# Autodesk Inventor assembly: Arm 2.0 Assembly
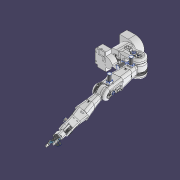
[picture p0: Inventor's stored thumbnail of the model, 180x180]
Saved by Autodesk Inventor 2017 SP1 (Build 210196100, 196)
## iProperties
Created: 2017-09-28
Part Number: Arm 2.0 Assembly
Document SubType Name: Assembly
Designer: Zach
Author: Zach
## Documents named in this file (62)
- C:\Users\Zach\Documents\GitHub\tr1\src\Body\Arm 2.0 Assembly\Arm 2.0 Assembly.iam
- C:\Users\Zach\Documents\GitHub\tr1\src\Body\Arm 2.0 Assembly\Steel Rod 8mm x 135mm.ipt
- C:\Users\Zach\Documents\GitHub\tr1\lib\22x8x8mm Bearing.ipt
- C:\Users\Zach\Documents\GitHub\tr1\src\Body\Arm 2.0 Assembly\AA004.ipt
- C:\Users\Zach\Documents\GitHub\tr1\lib\QS12MM250\QS12MM250.ipt
- C:\Users\Zach\Documents\GitHub\tr1\src\Body\Arm 2.0 Assembly\Steel Rod 8mm x 110mm.ipt
- C:\Users\Zach\Documents\GitHub\tr1\src\Body\Arm 2.0 Assembly\AA013.ipt
- C:\Users\Zach\Documents\GitHub\tr1\src\Body\Arm 2.0 Assembly\AA014.ipt
- C:\Users\Zach\Documents\GitHub\tr1\lib\12V DC Motor 378-1.ipt
- C:\Users\Zach\Documents\Inventor\Content Center Files\R2017\en-US\ISO 4017(1)\ISO 4017 - M5 x 20 - ISO.ipt
- C:\Users\Zach\Documents\GitHub\tr1\src\Body\Arm 2.0 Assembly\Steel Rod 8mm x 80mm.ipt
- C:\Users\Zach\Documents\GitHub\tr1\src\Body\Arm 2.0 Assembly\Gripper Assembly\Gripper B Assembly.iam
- C:\Users\Zach\Documents\GitHub\tr1\lib\8mm Hub.ipt
- C:\Users\Zach\Documents\GitHub\tr1\src\Body\Arm 2.0 Assembly\Arm 2.0 Assembly\Design Accelerator\Spur Gears5.iam
- C:\Users\Zach\Documents\GitHub\tr1\lib\4mm mounting hub.ipt
- C:\Users\Zach\Documents\GitHub\tr1\lib\6201RS\6201RS.ipt
- C:\Users\Zach\Documents\GitHub\tr1\lib\U51105\U51105.ipt
- C:\Users\Zach\Documents\GitHub\tr1\src\Body\Arm 2.0 Assembly\AA034.ipt
- C:\Users\Zach\Documents\GitHub\tr1\src\Body\Arm 2.0 Assembly\Arm 2.0 Assembly\Design Accelerator\Spur Gears6.iam
- C:\Users\Zach\Documents\GitHub\tr1\src\Body\Arm 2.0 Assembly\AA008c.ipt
- C:\Users\Zach\Documents\GitHub\tr1\src\Body\Arm 2.0 Assembly\Arm 2.0 Assembly\Design Accelerator\Spur Gears7.iam
- C:\Users\Zach\Documents\GitHub\tr1\src\Body\Arm 2.0 Assembly\AA036.ipt
- C:\Users\Zach\Documents\GitHub\tr1\src\Body\Arm 2.0 Assembly\AA037.ipt
- C:\Users\Zach\Documents\GitHub\tr1\src\Body\Arm 2.0 Assembly\AA016b.ipt
- C:\Users\Zach\Documents\GitHub\tr1\src\Body\Arm 2.0 Assembly\AA005b.ipt
- C:\Users\Zach\Documents\GitHub\tr1\src\Body\Arm 2.0 Assembly\AA006b.ipt
- C:\Users\Zach\Documents\GitHub\tr1\src\Body\Arm 2.0 Assembly\AA001c.ipt
- C:\Users\Zach\Documents\GitHub\tr1\src\Body\Arm 2.0 Assembly\Arm 2.0 Assembly\Design Accelerator\Spur Gears8.iam
- C:\Users\Zach\Documents\GitHub\tr1\src\Body\Arm 2.0 Assembly\Arm 2.0 Assembly\Design Accelerator\Spur Gears11.iam
- C:\Users\Zach\Documents\GitHub\tr1\src\Body\Arm 2.0 Assembly\Arm 2.0 Assembly\Design Accelerator\Spur Gears9.iam
- C:\Users\Zach\Documents\GitHub\tr1\src\Body\Arm 2.0 Assembly\AA010b.ipt
- C:\Users\Zach\Documents\GitHub\tr1\src\Body\Arm 2.0 Assembly\Arm 2.0 Assembly\Design Accelerator\Spur Gears10.iam
- C:\Users\Zach\Documents\GitHub\tr1\src\Body\Arm 2.0 Assembly\Arm 2.0 Assembly\Design Accelerator\Spur Gears12.iam
- C:\Users\Zach\Documents\GitHub\tr1\src\Body\Arm 2.0 Assembly\AA041.ipt
- C:\Users\Zach\Documents\Inventor\Content Center Files\R2017\en-US\ISO 7045  H\ISO 7045 - M3 x 8 - 4.8 - H - ISO.ipt
- C:\Users\Zach\Documents\GitHub\tr1\src\Body\Arm 2.0 Assembly\Arm 2.0 Assembly\Design Accelerator\Spur Gears13.iam
- C:\Users\Zach\Documents\GitHub\tr1\src\Body\Arm 2.0 Assembly\Arm 2.0 Assembly\Design Accelerator\Spur Gears16.iam
- C:\Users\Zach\Documents\GitHub\tr1\src\Body\Arm 2.0 Assembly\AA046.ipt
- C:\Users\Zach\Documents\GitHub\tr1\lib\MG995.ipt
- C:\Users\Zach\Documents\GitHub\tr1\lib\Servo Mounting Hub.ipt
- C:\Users\Zach\Documents\GitHub\tr1\src\Body\Arm 2.0 Assembly\AA047.ipt
- C:\Users\Zach\Documents\GitHub\tr1\src\Body\Arm 2.0 Assembly\AA048.ipt
- C:\Users\Zach\Documents\Inventor\Content Center Files\R2017\en-US\ISO 4018\ISO 4018 - M5 x 10.ipt
- C:\Users\Zach\Documents\Inventor\Content Center Files\R2017\en-US\ISO 4018\ISO 4018 - M5 x 25.ipt
- C:\Users\Zach\Documents\Inventor\Content Center Files\R2017\en-US\ISO 7045  H\ISO 7045 - M3 x 12 - 4.8 - H - ISO.ipt
- C:\Users\Zach\Documents\GitHub\tr1\src\Body\Arm 2.0 Assembly\AA049.ipt
- C:\Users\Zach\Documents\Inventor\Content Center Files\R2017\en-US\ISO 4018\ISO 4018 - M5 x 40.ipt
- C:\Users\Zach\Documents\Inventor\Content Center Files\R2017\en-US\ISO 4035(2)\ISO 4035 - M5 - ISO.ipt
- C:\Users\Zach\Documents\Inventor\Content Center Files\R2017\en-US\ISO 4018\ISO 4018 - M5 x 35.ipt
- C:\Users\Zach\Documents\Inventor\Content Center Files\R2017\en-US\ISO 4762(2)\ISO 4762 - M4 x 10ISO.ipt
- C:\Users\Zach\Documents\GitHub\tr1\src\Body\Arm 2.0 Assembly\AA050.ipt
- C:\Users\Zach\Documents\GitHub\tr1\lib\6mm Mounting Hub.ipt
- C:\Users\Zach\Documents\GitHub\tr1\src\Body\Arm 2.0 Assembly\AA035c.ipt
- C:\Users\Zach\Documents\GitHub\tr1\src\Body\Arm 2.0 Assembly\AA008d2.ipt
- C:\Users\Zach\Documents\GitHub\tr1\lib\TSINY TS-42GZ495.ipt
- C:\Users\Zach\Documents\GitHub\tr1\lib\EMS22XXX-D28-LSX.ipt
- C:\Users\Zach\Documents\GitHub\tr1\lib\6mm x 160mm D Shaft.ipt
- C:\Users\Zach\Documents\GitHub\tr1\src\Body\Arm 2.0 Assembly\AA051.ipt
- C:\Users\Zach\Documents\GitHub\tr1\src\Body\Arm 2.0 Assembly\AA052.ipt
- C:\Users\Zach\Documents\GitHub\tr1\src\Body\Arm 2.0 Assembly\AA045b.ipt
- C:\Users\Zach\Documents\GitHub\tr1\lib\6mm x 120mm D Shaft.ipt
- C:\Users\Zach\Documents\GitHub\tr1\src\Body\Arm 2.0 Assembly\AA053.ipt
## Components (215 placed, 61 different names)
1. AA001c:1 — Mate:554, Mate:555, Mate:556, Mate:560, Mate:562, Mate:563, Mate:564, Mate:565, Mate:566, Mate:567, Mate:576, Mate:578, Mate:581, Mate:592, Mate:602, Mate:895, Mate:905, Mate:906, Mate:1083, Mate:1084, Mate:1085, Mate:1086, Mate:1093, Angle:18, Mate:1095, Mate:1122, Mate:1261, Mate:1262, Mate:1263
2. AA004:1 — Mate:23, Mate:345, Mate:347, Mate:350, Mate:357, Mate:554, Mate:555, Mate:556, Mate:590, Mate:591, Mate:826
3. AA005b:1 — Mate:537, Mate:538, Mate:539, Mate:541, Mate:542, Mate:543, Mate:806, Mate:807, Mate:808, Mate:809, Mate:838, Mate:909, Mate:910
4. AA006b:1 — Mate:544, Mate:593, Mate:594, Mate:598, Mate:599, Mate:609, Mate:802, Mate:803, Mate:804, Mate:805, Mate:838, Mate:1088, Mate:1089, Angle:17, Mate:1233
5. AA008c:1 — Mate:451, Mate:616, Mate:1113, Mate:1114, Mate:1115, Mate:1125
6. AA008d2:1 — Mate:1104, Mate:1106, Mate:1107, Angle:22, Mate:1113, Mate:1114, Mate:1115, Mate:1124, Mate:1125, Mate:1157, Mate:1158, Mate:1159, Mate:1160, Mate:1161, Mate:1162, Mate:1163, Mate:1164, Mate:1165, Mate:1166, Mate:1170, Mate:1192, Mate:1193, Mate:1194, Mate:1195
7. AA010b:1 — Mate:616, Mate:620, Mate:621, Mate:624, Mate:625, Mate:626, Mate:628, Mate:630, Mate:642, Flush:20, Mate:648, Mate:650, Mate:948, Mate:1097, Mate:1098, Angle:21, Mate:1100, Mate:1101, Mate:1102, Mate:1126, Mate:1130, Mate:1152, Mate:1204, Mate:1237, Mate:1258, Mate:1259, Mate:1260
8. AA013:2 — Mate:142, Mate:143, Mate:144, Mate:145, Mate:146, Mate:147, Mate:563, Mate:564, Mate:565
9. AA014:2 — Mate:628, Mate:629, Mate:630, Mate:976, Mate:977, Mate:978, Mate:979, Mate:980, Mate:981
10. AA016b:1 — Mate:518, Mate:519, Mate:520, Mate:529, Mate:530, Mate:664, Mate:665, Mate:667, Mate:671, Mate:673, Mate:675, Mate:676, Mate:677, Mate:877, Mate:878, Mate:1206, Mate:1207, Angle:26
11. AA034:1 — Mate:529, Mate:534, Mate:535, Mate:879, Mate:880, Mate:881, Mate:882, Mate:883, Mate:884, Mate:885, Mate:886, Mate:964, Mate:965, Mate:966, Mate:967, Mate:968, Mate:969, Mate:970, Mate:971, Mate:972, Mate:973, Mate:974, Mate:975, Mate:1213, Mate:1256, Mate:1257
12. AA035c:1 — Mate:1076, Mate:1077, Mate:1167, Mate:1168, Mate:1169, Mate:1170, Mate:1171, Mate:1172, Mate:1173, Mate:1175, Angle:24, Angle:25, Mate:1176, Mate:1202, Mate:1203
13. AA036:1 — Mate:498, Mate:501, Mate:502, Mate:511, Mate:698, Mate:868, Mate:871, Mate:872, Mate:939, Mate:1197, Mate:1198, Mate:1199, Mate:1200
14. AA037:1 — Mate:501, Mate:502, Mate:514, Mate:515, Mate:516, Mate:518, Mate:519, Mate:520, Mate:530, Mate:664, Mate:665, Mate:698, Mate:866, Mate:867, Mate:873, Mate:874, Mate:875, Mate:876, Flush:25, Flush:26, Mate:950, Mate:951, Mate:952, Mate:953
15. AA041:1 — Mate:675, Mate:676, Mate:677, Mate:682, Mate:683, Mate:684, Mate:685, Mate:1250
16. AA045b:1 — Mate:1211, Mate:1212, Angle:27, Mate:1213, Mate:1214, Mate:1215, Mate:1216, Mate:1217, Mate:1218, Mate:1219, Flush:37, Mate:1221, Mate:1223, Mate:1224, Mate:1225, Mate:1227, Mate:1235, Mate:1264, Mate:1265
17. AA046:1 — Mate:727, Mate:728, Mate:731, Mate:735, Mate:736, Mate:737, Mate:752, Mate:756, Mate:757, Mate:758, Mate:759, Mate:760, Mate:761, Mate:762, Mate:763, Mate:1217
18. AA047:1 — Mate:735, Mate:736, Mate:737, Mate:738, Mate:739, Mate:740, Mate:753, Mate:754, Mate:755, Mate:800, Mate:801
19. AA048:1 — Mate:744, Mate:745, Mate:746, Mate:747, Mate:748, Mate:749
20. AA049:1 — Mate:783, Mate:786, Mate:787, Mate:788, Mate:789, Mate:790, Mate:791, Mate:1218
21. AA050:1 — Mate:994, Mate:995, Mate:999, Mate:1001, Mate:1002, Mate:1003, Mate:1004
22. AA051:1 — Mate:1196, Mate:1197
23. AA052:1 — Mate:1201, Mate:1202
24. AA053:1 — Mate:1258, Mate:1259, Mate:1260
25. AA053:3 — Mate:1261, Mate:1262, Mate:1263
26. Gripper B Assembly:1 [sub-assembly] — Mate:747, Mate:748, Mate:749
27. 22x8x8mm Bearing:1 — Mate:433, Mate:560
28. 22x8x8mm Bearing:2 — Mate:437, Mate:562
29. 22x8x8mm Bearing:3 — Mate:57, Mate:620, Mate:626
30. 22x8x8mm Bearing:4 — Mate:621, Mate:629, Mate:642
31. 22x8x8mm Bearing:5 — Mate:186, Mate:1265
32. 22x8x8mm Bearing:6 — Mate:187, Mate:1264
33. 22x8x8mm Bearing:7 — Mate:1247
34. 22x8x8mm Bearing:13 — Mate:451
35. QS12MM250:1 — Mate:23, Mate:344, Mate:346, Mate:348, Mate:354, Mate:537, Mate:544, Mate:593, Mate:594, Mate:597, Mate:1230
36. Steel Rod 8mm x 140mm:1 — Mate:433, Mate:437, Mate:476, Mate:575, Mate:651, Mate:1076, Mate:1122, Flush:35, Mate:1201
37. Steel Rod 8mm x 110mm:1 — Mate:57, Mate:491, Mate:498, Flush:20, Mate:649, Mate:1196, Mate:1204
38. Steel Rod 8mm x 80mm:1 — Mate:186, Mate:187, Mate:710, Mate:721, Mate:724, Mate:730, Mate:783, Mate:1216, Flush:37, Mate:1234
39. TSINY TS-42GZ495:3 — Mate:1104, Mate:1117, Mate:1135, Mate:1160, Mate:1161
40. TSINY TS-42GZ495:2 — Mate:1097, Mate:1098, Mate:1101, Mate:1102, Mate:1128, Mate:1129
41. TSINY TS-42GZ495:1 — Mate:1083, Mate:1084, Mate:1085, Mate:1086, Mate:1087
42. 12V DC Motor 378-1:3 — Mate:712, Mate:714, Mate:778, Mate:779, Mate:1224, Mate:1225
43. 12V DC Motor 378-1:4 — Mate:514, Mate:515, Mate:516, Mate:522
44. 12V DC Motor 378-1:6 — Mate:340, Mate:342, Mate:538, Mate:539, Mate:540, Mate:543, Mate:907, Mate:908
45. 6201RS:1 — Mate:346, Mate:347
46. 6201RS:2 — Mate:357, Mate:597
47. U51105:1 — Mate:348, Mate:349, Mate:542
48. U51105:2 — Mate:354, Mate:608, Mate:609, Mate:600
49. 6mm Mounting Hub:1 — Mate:1067, Mate:1069, Mate:1117, Mate:1136, Mate:1138, Mate:1139, Mate:1140, Flush:29, Mate:1243, Mate:1244
50. 6mm Mounting Hub:9 — Mate:1208, Flush:36, Mate:1209
51. 6mm Mounting Hub:7 — Mate:1185, Mate:1186, Mate:1188
52. 6mm Mounting Hub:8 — Mate:1189, Mate:1191
53. 6mm Mounting Hub:6 — Mate:1181, Mate:1183, Mate:1184
54. 6mm Mounting Hub:5 — Mate:1177, Mate:1178, Mate:1179
55. 6mm Mounting Hub:4 — Mate:1147, Mate:1148, Mate:1150, Mate:1152, Mate:1236, Mate:1238, Mate:1239, Mate:1240, Mate:1241, Mate:1242
56. 6mm Mounting Hub:2 — Mate:1090, Mate:1091
57. 8mm Hub:2 — Mate:534, Mate:535, Mate:1249, Mate:1254, Mate:1255
58. 8mm Hub:4 — Mate:580, Mate:581, Mate:582, Flush:35
59. 8mm Hub:6 — Mate:651, Mate:911, Mate:912, Mate:913, Mate:914, Mate:915, Mate:916, Mate:1203
60. 8mm Hub:7 — Mate:667, Mate:674, Flush:36, Mate:1248
61. 8mm Hub:8 — Mate:721, Mate:726, Mate:1220, Mate:1234
62. 8mm Hub:9 — Mate:727, Mate:728, Mate:730, Mate:756, Mate:764, Mate:765, Mate:766, Mate:767, Mate:768, Mate:769
63. 8mm Hub:10 — Mate:895, Mate:896, Mate:1087
64. 8mm Hub:11 — Mate:995, Mate:999, Mate:1005, Mate:1006, Mate:1245, Mate:1252, Mate:1253
65. 8mm Hub:12 — Mate:1011, Mate:1018, Mate:1019, Mate:1020, Mate:1132, Mate:1133, Mate:1137, Mate:1141, Mate:1142, Mate:1143, Mate:1144, Mate:1145, Mate:1146
66. 8mm Hub:13 — Mate:1129, Mate:1130, Mate:1131
67. 8mm Hub:14 — Mate:1198, Mate:1199, Mate:1200
68. 4mm mounting hub:1 — Mate:340, Mate:540, Mate:541, Mate:887
69. 4mm mounting hub:3 — Mate:522, Mate:994, Mate:997, Mate:1000, Mate:1001, Mate:1065, Mate:1066, Mate:1251
70. 4mm mounting hub:8 — Mate:714, Mate:716, Mate:782, Mate:1226
71. Servo Mounting Hub:1 — Mate:733, Mate:734, Mate:738, Mate:739, Mate:740, Mate:792, Mate:793, Mate:794, Mate:795, Mate:796, Mate:797, Mate:798, Mate:799
72. EMS22XXX-D28-LSX:1 — Mate:1088, Mate:1089, Angle:17, Mate:1090, Mate:1091, Mate:1181, Mate:1182, Mate:1232
73. EMS22XXX-D28-LSX:2 — Mate:1093, Angle:18, Mate:1095, Mate:1177, Mate:1180
74. EMS22XXX-D28-LSX:3 — Angle:21, Mate:1100, Mate:1126, Mate:1185, Mate:1187
75. EMS22XXX-D28-LSX:4 — Mate:1106, Mate:1107, Angle:22, Mate:1189, Mate:1190
76. EMS22XXX-D28-LSX:5 — Mate:1206, Mate:1207, Angle:26, Mate:1208, Mate:1210
77. EMS22XXX-D28-LSX:6 — Mate:1211, Mate:1212, Angle:27, Mate:1222, Mate:1228
78. AASG01 [sub-assembly] — Mate:342, Mate:344, Mate:345, Mate:349, Mate:350, Mate:810, Mate:811, Mate:812, Mate:813, Mate:814, Mate:815, Mate:816, Mate:817, Mate:818, Mate:819, Mate:820, Mate:821, Mate:887, Mate:888, Mate:889, Mate:890, Mate:891
79. AASG02 [sub-assembly] — Mate:476, Mate:566, Mate:567, Mate:602, Mate:839, Mate:841, Mate:842, Mate:843, Mate:844, Mate:845, Mate:896, Mate:897, Mate:898, Mate:899, Mate:900, Mate:901, Mate:902, Mate:1077
80. AASG03 [sub-assembly] — Mate:491, Mate:511, Mate:624, Mate:625, Mate:860, Mate:861, Mate:862, Mate:863, Mate:864, Mate:865, Mate:1128, Mate:1131
81. AASG04 [sub-assembly] — Mate:575, Mate:576, Mate:578, Mate:580, Mate:582, Mate:917, Mate:918, Mate:919, Mate:920, Mate:921, Mate:922, Mate:1178, Mate:1179, Mate:1180
82. AASG05 [sub-assembly] — Mate:590, Mate:591, Mate:592, Mate:608, Mate:822, Mate:823, Mate:824, Mate:825, Mate:827, Mate:828, Mate:829, Mate:830, Mate:831, Mate:832, Mate:833, Mate:1182, Mate:1183, Mate:1184, Mate:1230, Mate:1232, Mate:1233
83. AASG06 [sub-assembly] — Mate:1011, Mate:1067, Mate:1069, Mate:1124, Mate:1133, Mate:1134, Mate:1136, Mate:1137, Mate:1190, Mate:1191
84. AASG07 [sub-assembly] — Mate:648, Mate:649, Mate:650, Mate:958, Mate:959, Mate:960, Mate:961, Mate:962, Mate:963, Mate:1186, Mate:1187, Mate:1188
85. AASG08 [sub-assembly] — Mate:671, Mate:673, Mate:674, Mate:680, Mate:681, Mate:1209, Mate:1210
86. AASG09 [sub-assembly] — Mate:710, Mate:712, Mate:716, Mate:731, Mate:757, Mate:770, Mate:771, Mate:772, Mate:773, Mate:774, Mate:775, Mate:776, Mate:777, Mate:782, Mate:1223, Mate:1226, Mate:1227
87. AASG10 [sub-assembly] — Mate:724, Mate:726, Mate:1220, Mate:1221, Mate:1222, Mate:1229, Mate:1235
88. MG995:1 — Mate:733, Mate:734, Mate:744, Mate:745, Mate:746
89. ISO 7045 H M3 x 8 - 4.8 - H:1 — Mate:680, Mate:681
90. ISO 7045 H M3 x 8 - 4.8 - H:2 — Mate:682, Mate:685
91. ISO 7045 H M3 x 8 - 4.8 - H:3 — Mate:683, Mate:684
92. ISO 7045 H M3 x 8 - 4.8 - H:5 — Mate:778
93. ISO 7045 H M3 x 8 - 4.8 - H:6 — Mate:779
94. ISO 7045 H M3 x 8 - 4.8 - H:7 — Mate:795, Mate:799
95. ISO 7045 H M3 x 8 - 4.8 - H:8 — Mate:794, Mate:798
96. ISO 7045 H M3 x 8 - 4.8 - H:9 — Mate:792, Mate:796
97. ISO 7045 H M3 x 8 - 4.8 - H:10 — Mate:793, Mate:797
98. ISO 7045 H M3 x 8 - 4.8 - H:11 — Mate:800, Mate:801
99. ISO 7045 H M3 x 8 - 4.8 - H:13 — Mate:897, Mate:900
100. ISO 7045 H M3 x 8 - 4.8 - H:14 — Mate:898, Mate:901
101. ISO 7045 H M3 x 8 - 4.8 - H:15 — Mate:899, Mate:902
102. ISO 7045 H M3 x 8 - 4.8 - H:16 — Mate:908, Mate:910
103. ISO 7045 H M3 x 8 - 4.8 - H:17 — Mate:907, Mate:909
104. ISO 7045 H M3 x 8 - 4.8 - H:20 — Mate:951, Mate:953
105. ISO 7045 H M3 x 8 - 4.8 - H:21 — Mate:950, Mate:952
106. ISO 7045 H M3 x 8 - 4.8 - H:23 — Mate:1000, Mate:1066
107. ISO 7045 H M3 x 8 - 4.8 - H:22 — Mate:997, Mate:1065
108. ISO 7045 H M3 x 8 - 4.8 - H:24 — Mate:960, Mate:963
109. ISO 7045 H M3 x 8 - 4.8 - H:25 — Mate:958, Mate:962
110. ISO 7045 H M3 x 8 - 4.8 - H:26 — Mate:959, Mate:961
111. ISO 7045 H M3 x 8 - 4.8 - H:27 — Mate:965, Mate:972
112. ISO 7045 H M3 x 8 - 4.8 - H:28 — Mate:964, Mate:973
113. ISO 7045 H M3 x 8 - 4.8 - H:29 — Mate:966, Mate:971
114. ISO 7045 H M3 x 8 - 4.8 - H:30 — Mate:967, Mate:970, Mate:1256
115. ISO 7045 H M3 x 8 - 4.8 - H:31 — Mate:969, Mate:975
116. ISO 7045 H M3 x 8 - 4.8 - H:32 — Mate:968, Mate:974
117. ISO 7045 H M3 x 12 - 4.8 - H:1 — Mate:765, Mate:767
118. ISO 7045 H M3 x 12 - 4.8 - H:3 — Mate:764, Mate:769
119. ISO 7045 H M3 x 12 - 4.8 - H:2 — Mate:766, Mate:768
120. ISO 7045 H M3 x 12 - 4.8 - H:4 — Mate:770, Mate:775
121. ISO 7045 H M3 x 12 - 4.8 - H:5 — Mate:771, Mate:774
122. ISO 7045 H M3 x 12 - 4.8 - H:6 — Mate:773, Mate:777
123. ISO 7045 H M3 x 12 - 4.8 - H:7 — Mate:772, Mate:776
124. ISO 7045 H M3 x 12 - 4.8 - H:8 — Mate:889, Mate:890
125. ISO 7045 H M3 x 12 - 4.8 - H:9 — Mate:888, Mate:891
126. ISO 7045 H M3 x 12 - 4.8 - H:10 — Mate:911, Mate:914
127. ISO 7045 H M3 x 12 - 4.8 - H:11 — Mate:913, Mate:915
128. ISO 7045 H M3 x 12 - 4.8 - H:12 — Mate:912, Mate:916
129. ISO 7045 H M3 x 12 - 4.8 - H:13 — Mate:919, Mate:920
130. ISO 7045 H M3 x 12 - 4.8 - H:14 — Mate:917, Mate:921
131. ISO 7045 H M3 x 12 - 4.8 - H:15 — Mate:918, Mate:922
132. ISO 7045 H M3 x 12 - 4.8 - H:18 — Mate:1148, Mate:1240
133. ISO 7045 H M3 x 12 - 4.8 - H:19 — Mate:1236, Mate:1237, Mate:1238
134. ISO 7045 H M3 x 12 - 4.8 - H:20 — Mate:1150, Mate:1239
135. ISO 7045 H M3 x 12 - 4.8 - H:28 — Mate:1019, Mate:1140
136. ISO 7045 H M3 x 12 - 4.8 - H:29 — Mate:1018, Mate:1139
137. ISO 7045 H M3 x 12 - 4.8 - H:30 — Mate:1020, Mate:1138
138. ISO 7045 H M3 x 12 - 4.8 - H:25 — Mate:1002
139. ISO 7045 H M3 x 12 - 4.8 - H:26 — Mate:1003, Mate:1005
140. ISO 7045 H M3 x 12 - 4.8 - H:27 — Mate:1004, Mate:1006
141. ISO 7045 H M3 x 12 - 4.8 - H:31 — Mate:1141, Mate:1145
142. ISO 7045 H M3 x 12 - 4.8 - H:32 — Mate:1142, Mate:1146
143. ISO 7045 H M3 x 12 - 4.8 - H:33 — Mate:1143, Mate:1144
144. ISO 4762 M4 x 10:1 — Mate:905
145. ISO 4762 M4 x 10:2 — Mate:906
146. ISO 4762 M4 x 10:4 — Mate:948
147. ISO 4035 M5:1 — Mate:1167, Mate:1168
148. ISO 4035 M5:2 — Mate:852, Mate:1176
149. ISO 4035 M5:3 — Mate:869, Mate:872
150. ISO 4035 M5:4 — Mate:870, Mate:871
151. ISO 4035 M5:5 — Mate:985
152. ISO 4035 M5:6 — Mate:984
153. ISO 4035 M5:7 — Mate:989
154. ISO 4035 M5:8 — Mate:988
155. ISO 4035 M5:9 — Mate:1174, Mate:1175, Angle:24
156. ISO 4035 M5:10 — Mate:1027, Mate:1173, Angle:25
157. ISO 4018 M5 x 10:1 — Mate:754, Mate:755
158. ISO 4018 M5 x 10:2 — Mate:752, Mate:753
159. ISO 4018 M5 x 10:3 — Mate:787, Mate:790
160. ISO 4018 M5 x 10:4 — Mate:788, Mate:791
161. ISO 4018 M5 x 10:5 — Mate:786, Mate:789, Mate:1219
162. ISO 4017 M5 x 20:1 — Mate:146, Mate:147
163. ISO 4017 M5 x 20:2 — Mate:144, Mate:145
164. ISO 4017 M5 x 20:3 — Mate:142, Mate:143
165. ISO 4017 M5 x 20:4 — Mate:978, Mate:980
166. ISO 4017 M5 x 20:5 — Mate:977, Mate:979
167. ISO 4017 M5 x 20:6 — Mate:976, Mate:981
168. ISO 4018 M5 x 25:1 — Mate:758, Mate:761
169. ISO 4018 M5 x 25:2 — Mate:759, Mate:763
170. ISO 4018 M5 x 25:3 — Mate:760, Mate:762
171. ISO 4018 M5 x 25:7 — Mate:802, Mate:803
172. ISO 4018 M5 x 25:8 — Mate:804, Mate:805
173. ISO 4018 M5 x 25:9 — Mate:806, Mate:808
174. ISO 4018 M5 x 25:10 — Mate:807, Mate:809
175. ISO 4018 M5 x 25:11 — Mate:812, Mate:820
176. ISO 4018 M5 x 25:12 — Mate:810, Mate:816
177. ISO 4018 M5 x 25:13 — Mate:811, Mate:821
178. ISO 4018 M5 x 25:14 — Mate:814, Mate:817
179. ISO 4018 M5 x 25:15 — Mate:813, Mate:819
180. ISO 4018 M5 x 25:16 — Mate:815, Mate:818
181. ISO 4018 M5 x 25:17 — Mate:823, Mate:831
182. ISO 4018 M5 x 25:18 — Mate:824, Mate:829
183. ISO 4018 M5 x 25:19 — Mate:825, Mate:832
184. ISO 4018 M5 x 25:20 — Mate:827, Mate:828
185. ISO 4018 M5 x 25:21 — Mate:826, Mate:833
186. ISO 4018 M5 x 25:22 — Mate:822, Mate:830
187. ISO 4018 M5 x 25:23
188. ISO 4018 M5 x 25:24
189. ISO 4018 M5 x 25:25 — Mate:839, Mate:845
190. ISO 4018 M5 x 25:27 — Mate:841, Mate:844
191. ISO 4018 M5 x 25:28 — Mate:842, Mate:843
192. ISO 4018 M5 x 25:29 — Mate:1157, Mate:1159
193. ISO 4018 M5 x 25:30 — Mate:1192, Mate:1193
194. ISO 4018 M5 x 25:31 — Mate:1194, Mate:1195
195. ISO 4018 M5 x 25:32 — Mate:1158
196. ISO 4018 M5 x 25:33 — Mate:860, Mate:865, Mate:939
197. ISO 4018 M5 x 25:34 — Mate:862, Mate:863
198. ISO 4018 M5 x 25:35 — Mate:861, Mate:864
199. ISO 4018 M5 x 25:36 — Mate:876, Mate:878
200. ISO 4018 M5 x 25:37 — Mate:875, Mate:877
201. ISO 4018 M5 x 25:38 — Mate:874, Flush:26
202. ISO 4018 M5 x 25:39 — Mate:873, Flush:25
203. ISO 4018 M5 x 25:40 — Mate:882, Mate:883, Mate:984
204. ISO 4018 M5 x 25:41 — Mate:880, Mate:886, Mate:988, Mate:1214
205. ISO 4018 M5 x 25:42 — Mate:879, Mate:885, Mate:985
206. ISO 4018 M5 x 25:43 — Mate:881, Mate:884, Mate:989, Mate:1215
207. ISO 4018 M5 x 35:1 — Mate:866, Mate:867, Flush:24, Mate:869
208. ISO 4018 M5 x 35:2 — Mate:868, Flush:24, Mate:870
209. ISO 4018 M5 x 40:1 — Mate:1162, Mate:1169
210. ISO 4018 M5 x 40:2 — Mate:852, Mate:1163, Mate:1166
211. ISO 4018 M5 x 40:3 — Mate:1027, Mate:1165, Mate:1172
212. ISO 4018 M5 x 40:4 — Mate:1164, Mate:1171, Mate:1174
213. 6mm x 160mm D Shaft:1 — Mate:1132, Mate:1134, Mate:1135, Flush:29, Mate:1147, Mate:1241, Mate:1242, Mate:1243, Mate:1244
214. 6mm Mounting Hub:10 — Mate:1228, Mate:1229
215. 6mm x 120mm D Shaft:1 — Mate:1245, Mate:1247, Mate:1248, Mate:1249, Mate:1250, Mate:1251, Mate:1252, Mate:1253, Mate:1254, Mate:1255, Mate:1257
## Relationships (504: Mate 488, Flush 8, Angle 8)
- Mate:23: AA004:1 ↔ QS12MM250:1
- Mate:57: 22x8x8mm Bearing:3 ↔ Steel Rod 8mm x 110mm:1
- Mate:142: AA013:2 ↔ ISO 4017 M5 x 20:3
- Mate:143: AA013:2 ↔ ISO 4017 M5 x 20:3
- Mate:144: AA013:2 ↔ ISO 4017 M5 x 20:2
- Mate:145: AA013:2 ↔ ISO 4017 M5 x 20:2
- Mate:146: AA013:2 ↔ ISO 4017 M5 x 20:1
- Mate:147: AA013:2 ↔ ISO 4017 M5 x 20:1
- Mate:186: 22x8x8mm Bearing:5 ↔ Steel Rod 8mm x 80mm:1
- Mate:187: 22x8x8mm Bearing:6 ↔ Steel Rod 8mm x 80mm:1
- Mate:340: 12V DC Motor 378-1:6 ↔ 4mm mounting hub:1
- Mate:342: 12V DC Motor 378-1:6 ↔ AASG01
- Mate:344: QS12MM250:1 ↔ AASG01
- Mate:345: AA004:1 ↔ AASG01
- Mate:346: QS12MM250:1 ↔ 6201RS:1
- Mate:347: AA004:1 ↔ 6201RS:1
- Mate:348: QS12MM250:1 ↔ U51105:1
- Mate:349: U51105:1 ↔ AASG01
- Mate:350: AA004:1 ↔ AASG01
- Mate:354: QS12MM250:1 ↔ U51105:2
- Mate:357: AA004:1 ↔ 6201RS:2
- Mate:433: 22x8x8mm Bearing:1 ↔ Steel Rod 8mm x 140mm:1
- Mate:437: 22x8x8mm Bearing:2 ↔ Steel Rod 8mm x 140mm:1
- Mate:451: AA008c:1 ↔ 22x8x8mm Bearing:13
- Mate:476: Steel Rod 8mm x 140mm:1 ↔ AASG02
- Mate:491: Steel Rod 8mm x 110mm:1 ↔ AASG03
- Mate:498: AA036:1 ↔ Steel Rod 8mm x 110mm:1
- Mate:501: AA036:1 ↔ AA037:1
- Mate:502: AA036:1 ↔ AA037:1
- Mate:511: AA036:1 ↔ AASG03
- Mate:514: AA037:1 ↔ 12V DC Motor 378-1:4
- Mate:515: AA037:1 ↔ 12V DC Motor 378-1:4
- Mate:516: AA037:1 ↔ 12V DC Motor 378-1:4
- Mate:518: AA016b:1 ↔ AA037:1
- Mate:519: AA016b:1 ↔ AA037:1
- Mate:520: AA016b:1 ↔ AA037:1
- Mate:522: 12V DC Motor 378-1:4 ↔ 4mm mounting hub:3
- Mate:529: AA016b:1 ↔ AA034:1
- Mate:530: AA016b:1 ↔ AA037:1
- Mate:534: AA034:1 ↔ 8mm Hub:2
- Mate:535: AA034:1 ↔ 8mm Hub:2
- Mate:537: AA005b:1 ↔ QS12MM250:1
- Mate:538: AA005b:1 ↔ 12V DC Motor 378-1:6
- Mate:539: AA005b:1 ↔ 12V DC Motor 378-1:6
- Mate:540: 12V DC Motor 378-1:6 ↔ 4mm mounting hub:1
- Mate:541: AA005b:1 ↔ 4mm mounting hub:1
- Mate:542: AA005b:1 ↔ U51105:1
- Mate:543: AA005b:1 ↔ 12V DC Motor 378-1:6
- Mate:544: AA006b:1 ↔ QS12MM250:1
- Mate:554: AA001c:1 ↔ AA004:1
- Mate:555: AA001c:1 ↔ AA004:1
- Mate:556: AA001c:1 ↔ AA004:1
- Mate:560: AA001c:1 ↔ 22x8x8mm Bearing:1
- Mate:562: AA001c:1 ↔ 22x8x8mm Bearing:2
- Mate:563: AA001c:1 ↔ AA013:2
- Mate:564: AA001c:1 ↔ AA013:2
- Mate:565: AA001c:1 ↔ AA013:2
- Mate:566: AA001c:1 ↔ AASG02
- Mate:567 (1 mm): AA001c:1 ↔ AASG02
- Mate:575: Steel Rod 8mm x 140mm:1 ↔ AASG04
- Mate:576: AA001c:1 ↔ AASG04
- Mate:578: AA001c:1 ↔ AASG04
- Mate:580: 8mm Hub:4 ↔ AASG04
- Mate:581: AA001c:1 ↔ 8mm Hub:4
- Mate:582: 8mm Hub:4 ↔ AASG04
- Mate:590: AA004:1 ↔ AASG05
- Mate:591: AA004:1 ↔ AASG05
- Mate:592: AA001c:1 ↔ AASG05
- Mate:593: AA006b:1 ↔ QS12MM250:1
- Mate:594: AA006b:1 ↔ QS12MM250:1
- Mate:597: QS12MM250:1 ↔ 6201RS:2
- Mate:598: AA006b:1
- Mate:599: AA006b:1
- Mate:600: U51105:2
- Mate:602 (2.5 mm): AA001c:1 ↔ AASG02
- Mate:608: U51105:2 ↔ AASG05
- Mate:609: AA006b:1 ↔ U51105:2
- Mate:616: AA008c:1 ↔ AA010b:1
- Mate:620: AA010b:1 ↔ 22x8x8mm Bearing:3
- Mate:621: AA010b:1 ↔ 22x8x8mm Bearing:4
- Mate:624: AA010b:1 ↔ AASG03
- Mate:625: AA010b:1 ↔ AASG03
- Flush:20 (0.5 mm): AA010b:1 ↔ Steel Rod 8mm x 110mm:1
- Mate:626: AA010b:1 ↔ 22x8x8mm Bearing:3
- Mate:628: AA010b:1 ↔ AA014:2
- Mate:629: AA014:2 ↔ 22x8x8mm Bearing:4
- Mate:630: AA010b:1 ↔ AA014:2
- Mate:642: AA010b:1 ↔ 22x8x8mm Bearing:4
- Mate:648: AA010b:1 ↔ AASG07
- Mate:649: Steel Rod 8mm x 110mm:1 ↔ AASG07
- Mate:650: AA010b:1 ↔ AASG07
- Mate:651: Steel Rod 8mm x 140mm:1 ↔ 8mm Hub:6
- Mate:664: AA016b:1 ↔ AA037:1
- Mate:665: AA016b:1 ↔ AA037:1
- Mate:667: AA016b:1 ↔ 8mm Hub:7
- Mate:671: AA016b:1 ↔ AASG08
- Mate:673: AA016b:1 ↔ AASG08
- Mate:674: 8mm Hub:7 ↔ AASG08
- Mate:675: AA016b:1 ↔ AA041:1
- Mate:676: AA016b:1 ↔ AA041:1
- Mate:677: AA016b:1 ↔ AA041:1
- Mate:680: AASG08 ↔ ISO 7045 H M3 x 8 - 4.8 - H:1
- Mate:681: AASG08 ↔ ISO 7045 H M3 x 8 - 4.8 - H:1
- Mate:682: AA041:1 ↔ ISO 7045 H M3 x 8 - 4.8 - H:2
- Mate:683: AA041:1 ↔ ISO 7045 H M3 x 8 - 4.8 - H:3
- Mate:684: AA041:1 ↔ ISO 7045 H M3 x 8 - 4.8 - H:3
- Mate:685: AA041:1 ↔ ISO 7045 H M3 x 8 - 4.8 - H:2
- Mate:698: AA036:1 ↔ AA037:1
- Mate:710: Steel Rod 8mm x 80mm:1 ↔ AASG09
- Mate:712: 12V DC Motor 378-1:3 ↔ AASG09
- Mate:714: 12V DC Motor 378-1:3 ↔ 4mm mounting hub:8
- Mate:716: 4mm mounting hub:8 ↔ AASG09
- Mate:721: Steel Rod 8mm x 80mm:1 ↔ 8mm Hub:8
- Mate:724: Steel Rod 8mm x 80mm:1 ↔ AASG10
- Mate:726: 8mm Hub:8 ↔ AASG10
- Mate:727: AA046:1 ↔ 8mm Hub:9
- Mate:728: AA046:1 ↔ 8mm Hub:9
- Mate:730: Steel Rod 8mm x 80mm:1 ↔ 8mm Hub:9
- Mate:731: AA046:1 ↔ AASG09
- Mate:733: Servo Mounting Hub:1 ↔ MG995:1
- Mate:734: Servo Mounting Hub:1 ↔ MG995:1
- Mate:735: AA046:1 ↔ AA047:1
- Mate:736: AA046:1 ↔ AA047:1
- Mate:737: AA046:1 ↔ AA047:1
- Mate:738: AA047:1 ↔ Servo Mounting Hub:1
- Mate:739: AA047:1 ↔ Servo Mounting Hub:1
- Mate:740: AA047:1 ↔ Servo Mounting Hub:1
- Mate:744: AA048:1 ↔ MG995:1
- Mate:745 (0.5 mm): AA048:1 ↔ MG995:1
- Mate:746 (0.5 mm): AA048:1 ↔ MG995:1
- Mate:747: AA048:1 ↔ Gripper B Assembly:1
- Mate:748: AA048:1 ↔ Gripper B Assembly:1
- Mate:749: AA048:1 ↔ Gripper B Assembly:1
- Mate:752: AA046:1 ↔ ISO 4018 M5 x 10:2
- Mate:753: AA047:1 ↔ ISO 4018 M5 x 10:2
- Mate:754: AA047:1 ↔ ISO 4018 M5 x 10:1
- Mate:755: AA047:1 ↔ ISO 4018 M5 x 10:1
- Mate:756: AA046:1 ↔ 8mm Hub:9
- Mate:757: AA046:1 ↔ AASG09
- Mate:758: AA046:1 ↔ ISO 4018 M5 x 25:1
- Mate:759: AA046:1 ↔ ISO 4018 M5 x 25:2
- Mate:760: AA046:1 ↔ ISO 4018 M5 x 25:3
- Mate:761: AA046:1 ↔ ISO 4018 M5 x 25:1
- Mate:762: AA046:1 ↔ ISO 4018 M5 x 25:3
- Mate:763: AA046:1 ↔ ISO 4018 M5 x 25:2
- Mate:764: 8mm Hub:9 ↔ ISO 7045 H M3 x 12 - 4.8 - H:3
- Mate:765: 8mm Hub:9 ↔ ISO 7045 H M3 x 12 - 4.8 - H:1
- Mate:766: 8mm Hub:9 ↔ ISO 7045 H M3 x 12 - 4.8 - H:2
- Mate:767: 8mm Hub:9 ↔ ISO 7045 H M3 x 12 - 4.8 - H:1
- Mate:768: 8mm Hub:9 ↔ ISO 7045 H M3 x 12 - 4.8 - H:2
- Mate:769: 8mm Hub:9 ↔ ISO 7045 H M3 x 12 - 4.8 - H:3
- Mate:770: AASG09 ↔ ISO 7045 H M3 x 12 - 4.8 - H:4
- Mate:771: AASG09 ↔ ISO 7045 H M3 x 12 - 4.8 - H:5
- Mate:772: AASG09 ↔ ISO 7045 H M3 x 12 - 4.8 - H:7
- Mate:773: AASG09 ↔ ISO 7045 H M3 x 12 - 4.8 - H:6
- Mate:774: AASG09 ↔ ISO 7045 H M3 x 12 - 4.8 - H:5
- Mate:775: AASG09 ↔ ISO 7045 H M3 x 12 - 4.8 - H:4
- Mate:776: AASG09 ↔ ISO 7045 H M3 x 12 - 4.8 - H:7
- Mate:777: AASG09 ↔ ISO 7045 H M3 x 12 - 4.8 - H:6
- Mate:778: 12V DC Motor 378-1:3 ↔ ISO 7045 H M3 x 8 - 4.8 - H:5
- Mate:779: 12V DC Motor 378-1:3 ↔ ISO 7045 H M3 x 8 - 4.8 - H:6
- Mate:782: 4mm mounting hub:8 ↔ AASG09
- Mate:783: AA049:1 ↔ Steel Rod 8mm x 80mm:1
- Mate:786: AA049:1 ↔ ISO 4018 M5 x 10:5
- Mate:787: AA049:1 ↔ ISO 4018 M5 x 10:3
- Mate:788: AA049:1 ↔ ISO 4018 M5 x 10:4
- Mate:789: AA049:1 ↔ ISO 4018 M5 x 10:5
- Mate:790: AA049:1 ↔ ISO 4018 M5 x 10:3
- Mate:791: AA049:1 ↔ ISO 4018 M5 x 10:4
- Mate:792: Servo Mounting Hub:1 ↔ ISO 7045 H M3 x 8 - 4.8 - H:9
- Mate:793: Servo Mounting Hub:1 ↔ ISO 7045 H M3 x 8 - 4.8 - H:10
- Mate:794: Servo Mounting Hub:1 ↔ ISO 7045 H M3 x 8 - 4.8 - H:8
- Mate:795: Servo Mounting Hub:1 ↔ ISO 7045 H M3 x 8 - 4.8 - H:7
- Mate:796: Servo Mounting Hub:1 ↔ ISO 7045 H M3 x 8 - 4.8 - H:9
- Mate:797: Servo Mounting Hub:1 ↔ ISO 7045 H M3 x 8 - 4.8 - H:10
- Mate:798: Servo Mounting Hub:1 ↔ ISO 7045 H M3 x 8 - 4.8 - H:8
- Mate:799: Servo Mounting Hub:1 ↔ ISO 7045 H M3 x 8 - 4.8 - H:7
- Mate:800: AA047:1 ↔ ISO 7045 H M3 x 8 - 4.8 - H:11
- Mate:801: AA047:1 ↔ ISO 7045 H M3 x 8 - 4.8 - H:11
- Mate:802: AA006b:1 ↔ ISO 4018 M5 x 25:7
- Mate:803: AA006b:1 ↔ ISO 4018 M5 x 25:7
- Mate:804: AA006b:1 ↔ ISO 4018 M5 x 25:8
- Mate:805: AA006b:1 ↔ ISO 4018 M5 x 25:8
- Mate:806: AA005b:1 ↔ ISO 4018 M5 x 25:9
- Mate:807: AA005b:1 ↔ ISO 4018 M5 x 25:10
- Mate:808: AA005b:1 ↔ ISO 4018 M5 x 25:9
- Mate:809: AA005b:1 ↔ ISO 4018 M5 x 25:10
- Mate:810: AASG01 ↔ ISO 4018 M5 x 25:12
- Mate:811: AASG01 ↔ ISO 4018 M5 x 25:13
- Mate:812: AASG01 ↔ ISO 4018 M5 x 25:11
- Mate:813: AASG01 ↔ ISO 4018 M5 x 25:15
- Mate:814: AASG01 ↔ ISO 4018 M5 x 25:14
- Mate:815: AASG01 ↔ ISO 4018 M5 x 25:16
- Mate:816: AASG01 ↔ ISO 4018 M5 x 25:12
- Mate:817: AASG01 ↔ ISO 4018 M5 x 25:14
- Mate:818: AASG01 ↔ ISO 4018 M5 x 25:16
- Mate:819: AASG01 ↔ ISO 4018 M5 x 25:15
- Mate:820: AASG01 ↔ ISO 4018 M5 x 25:11
- Mate:821: AASG01 ↔ ISO 4018 M5 x 25:13
- Mate:822: AASG05 ↔ ISO 4018 M5 x 25:22
- Mate:823: AASG05 ↔ ISO 4018 M5 x 25:17
- Mate:824: AASG05 ↔ ISO 4018 M5 x 25:18
- Mate:825: AASG05 ↔ ISO 4018 M5 x 25:19
- Mate:826: AA004:1 ↔ ISO 4018 M5 x 25:21
- Mate:827: AASG05 ↔ ISO 4018 M5 x 25:20
- Mate:828: AASG05 ↔ ISO 4018 M5 x 25:20
- Mate:829: AASG05 ↔ ISO 4018 M5 x 25:18
- Mate:830: AASG05 ↔ ISO 4018 M5 x 25:22
- Mate:831: AASG05 ↔ ISO 4018 M5 x 25:17
- Mate:832: AASG05 ↔ ISO 4018 M5 x 25:19
- Mate:833: AASG05 ↔ ISO 4018 M5 x 25:21
- Mate:838: AA005b:1 ↔ AA006b:1
- Mate:839: AASG02 ↔ ISO 4018 M5 x 25:25
- Mate:841: AASG02 ↔ ISO 4018 M5 x 25:27
- Mate:842: AASG02 ↔ ISO 4018 M5 x 25:28
- Mate:843: AASG02 ↔ ISO 4018 M5 x 25:28
- Mate:844: AASG02 ↔ ISO 4018 M5 x 25:27
- Mate:845: AASG02 ↔ ISO 4018 M5 x 25:25
- Mate:852: ISO 4035 M5:2 ↔ ISO 4018 M5 x 40:2
- Mate:860: AASG03 ↔ ISO 4018 M5 x 25:33
- Mate:861: AASG03 ↔ ISO 4018 M5 x 25:35
- Mate:862: AASG03 ↔ ISO 4018 M5 x 25:34
- Mate:863: AASG03 ↔ ISO 4018 M5 x 25:34
- Mate:864: AASG03 ↔ ISO 4018 M5 x 25:35
- Mate:865: AASG03 ↔ ISO 4018 M5 x 25:33
- Mate:866: AA037:1 ↔ ISO 4018 M5 x 35:1
- Mate:867: AA037:1 ↔ ISO 4018 M5 x 35:1
- Mate:868: AA036:1 ↔ ISO 4018 M5 x 35:2
- Flush:24: ISO 4018 M5 x 35:1 ↔ ISO 4018 M5 x 35:2
- Mate:869: ISO 4035 M5:3 ↔ ISO 4018 M5 x 35:1
- Mate:870: ISO 4035 M5:4 ↔ ISO 4018 M5 x 35:2
- Mate:871: AA036:1 ↔ ISO 4035 M5:4
- Mate:872: AA036:1 ↔ ISO 4035 M5:3
- Mate:873: AA037:1 ↔ ISO 4018 M5 x 25:39
- Mate:874: AA037:1 ↔ ISO 4018 M5 x 25:38
- Mate:875: AA037:1 ↔ ISO 4018 M5 x 25:37
- Mate:876: AA037:1 ↔ ISO 4018 M5 x 25:36
- Flush:25 (-9 mm): AA037:1 ↔ ISO 4018 M5 x 25:39
- Flush:26 (9 mm): AA037:1 ↔ ISO 4018 M5 x 25:38
- Mate:877: AA016b:1 ↔ ISO 4018 M5 x 25:37
- Mate:878: AA016b:1 ↔ ISO 4018 M5 x 25:36
- Mate:879: AA034:1 ↔ ISO 4018 M5 x 25:42
- Mate:880: AA034:1 ↔ ISO 4018 M5 x 25:41
- Mate:881: AA034:1 ↔ ISO 4018 M5 x 25:43
- Mate:882: AA034:1 ↔ ISO 4018 M5 x 25:40
- Mate:883: AA034:1 ↔ ISO 4018 M5 x 25:40
- Mate:884: AA034:1 ↔ ISO 4018 M5 x 25:43
- Mate:885: AA034:1 ↔ ISO 4018 M5 x 25:42
- Mate:886: AA034:1 ↔ ISO 4018 M5 x 25:41
- Mate:887: 4mm mounting hub:1 ↔ AASG01
- Mate:888: AASG01 ↔ ISO 7045 H M3 x 12 - 4.8 - H:9
- Mate:889: AASG01 ↔ ISO 7045 H M3 x 12 - 4.8 - H:8
- Mate:890: AASG01 ↔ ISO 7045 H M3 x 12 - 4.8 - H:8
- Mate:891: AASG01 ↔ ISO 7045 H M3 x 12 - 4.8 - H:9
- Mate:895: AA001c:1 ↔ 8mm Hub:10
- Mate:896: 8mm Hub:10 ↔ AASG02
- Mate:897: AASG02 ↔ ISO 7045 H M3 x 8 - 4.8 - H:13
- Mate:898: AASG02 ↔ ISO 7045 H M3 x 8 - 4.8 - H:14
- Mate:899: AASG02 ↔ ISO 7045 H M3 x 8 - 4.8 - H:15
- Mate:900: AASG02 ↔ ISO 7045 H M3 x 8 - 4.8 - H:13
- Mate:901: AASG02 ↔ ISO 7045 H M3 x 8 - 4.8 - H:14
- Mate:902: AASG02 ↔ ISO 7045 H M3 x 8 - 4.8 - H:15
- Mate:905: AA001c:1 ↔ ISO 4762 M4 x 10:1
- Mate:906: AA001c:1 ↔ ISO 4762 M4 x 10:2
- Mate:907: 12V DC Motor 378-1:6 ↔ ISO 7045 H M3 x 8 - 4.8 - H:17
- Mate:908: 12V DC Motor 378-1:6 ↔ ISO 7045 H M3 x 8 - 4.8 - H:16
- Mate:909: AA005b:1 ↔ ISO 7045 H M3 x 8 - 4.8 - H:17
- Mate:910: AA005b:1 ↔ ISO 7045 H M3 x 8 - 4.8 - H:16
- Mate:911: 8mm Hub:6 ↔ ISO 7045 H M3 x 12 - 4.8 - H:10
- Mate:912: 8mm Hub:6 ↔ ISO 7045 H M3 x 12 - 4.8 - H:12
- Mate:913: 8mm Hub:6 ↔ ISO 7045 H M3 x 12 - 4.8 - H:11
- Mate:914: 8mm Hub:6 ↔ ISO 7045 H M3 x 12 - 4.8 - H:10
- Mate:915: 8mm Hub:6 ↔ ISO 7045 H M3 x 12 - 4.8 - H:11
- Mate:916: 8mm Hub:6 ↔ ISO 7045 H M3 x 12 - 4.8 - H:12
- Mate:917: AASG04 ↔ ISO 7045 H M3 x 12 - 4.8 - H:14
- Mate:918: AASG04 ↔ ISO 7045 H M3 x 12 - 4.8 - H:15
- Mate:919: AASG04 ↔ ISO 7045 H M3 x 12 - 4.8 - H:13
- Mate:920: AASG04 ↔ ISO 7045 H M3 x 12 - 4.8 - H:13
- Mate:921: AASG04 ↔ ISO 7045 H M3 x 12 - 4.8 - H:14
- Mate:922: AASG04 ↔ ISO 7045 H M3 x 12 - 4.8 - H:15
- Mate:939: AA036:1 ↔ ISO 4018 M5 x 25:33
- Mate:948: AA010b:1 ↔ ISO 4762 M4 x 10:4
- Mate:950: AA037:1 ↔ ISO 7045 H M3 x 8 - 4.8 - H:21
- Mate:951: AA037:1 ↔ ISO 7045 H M3 x 8 - 4.8 - H:20
- Mate:952: AA037:1 ↔ ISO 7045 H M3 x 8 - 4.8 - H:21
- Mate:953: AA037:1 ↔ ISO 7045 H M3 x 8 - 4.8 - H:20
- Mate:958: AASG07 ↔ ISO 7045 H M3 x 8 - 4.8 - H:25
- Mate:959: AASG07 ↔ ISO 7045 H M3 x 8 - 4.8 - H:26
- Mate:960: AASG07 ↔ ISO 7045 H M3 x 8 - 4.8 - H:24
- Mate:961: AASG07 ↔ ISO 7045 H M3 x 8 - 4.8 - H:26
- Mate:962: AASG07 ↔ ISO 7045 H M3 x 8 - 4.8 - H:25
- Mate:963: AASG07 ↔ ISO 7045 H M3 x 8 - 4.8 - H:24
- Mate:964: AA034:1 ↔ ISO 7045 H M3 x 8 - 4.8 - H:28
- Mate:965: AA034:1 ↔ ISO 7045 H M3 x 8 - 4.8 - H:27
- Mate:966: AA034:1 ↔ ISO 7045 H M3 x 8 - 4.8 - H:29
- Mate:967: AA034:1 ↔ ISO 7045 H M3 x 8 - 4.8 - H:30
- Mate:968: AA034:1 ↔ ISO 7045 H M3 x 8 - 4.8 - H:32
- Mate:969: AA034:1 ↔ ISO 7045 H M3 x 8 - 4.8 - H:31
- Mate:970: AA034:1 ↔ ISO 7045 H M3 x 8 - 4.8 - H:30
- Mate:971: AA034:1 ↔ ISO 7045 H M3 x 8 - 4.8 - H:29
- Mate:972: AA034:1 ↔ ISO 7045 H M3 x 8 - 4.8 - H:27
- Mate:973: AA034:1 ↔ ISO 7045 H M3 x 8 - 4.8 - H:28
- Mate:974: AA034:1 ↔ ISO 7045 H M3 x 8 - 4.8 - H:32
- Mate:975: AA034:1 ↔ ISO 7045 H M3 x 8 - 4.8 - H:31
- Mate:976: AA014:2 ↔ ISO 4017 M5 x 20:6
- Mate:977: AA014:2 ↔ ISO 4017 M5 x 20:5
- Mate:978: AA014:2 ↔ ISO 4017 M5 x 20:4
- Mate:979: AA014:2 ↔ ISO 4017 M5 x 20:5
- Mate:980: AA014:2 ↔ ISO 4017 M5 x 20:4
- Mate:981: AA014:2 ↔ ISO 4017 M5 x 20:6
- Mate:984: ISO 4035 M5:6 ↔ ISO 4018 M5 x 25:40
- Mate:985: ISO 4035 M5:5 ↔ ISO 4018 M5 x 25:42
- Mate:988: ISO 4035 M5:8 ↔ ISO 4018 M5 x 25:41
- Mate:989: ISO 4035 M5:7 ↔ ISO 4018 M5 x 25:43
- Mate:994: AA050:1 ↔ 4mm mounting hub:3
- Mate:995: AA050:1 ↔ 8mm Hub:11
- Mate:997: 4mm mounting hub:3 ↔ ISO 7045 H M3 x 8 - 4.8 - H:22
- Mate:999: AA050:1 ↔ 8mm Hub:11
- Mate:1000: 4mm mounting hub:3 ↔ ISO 7045 H M3 x 8 - 4.8 - H:23
- Mate:1001: AA050:1 ↔ 4mm mounting hub:3
- Mate:1002: AA050:1 ↔ ISO 7045 H M3 x 12 - 4.8 - H:25
- Mate:1003: AA050:1 ↔ ISO 7045 H M3 x 12 - 4.8 - H:26
- Mate:1004: AA050:1 ↔ ISO 7045 H M3 x 12 - 4.8 - H:27
- Mate:1005: 8mm Hub:11 ↔ ISO 7045 H M3 x 12 - 4.8 - H:26
- Mate:1006: 8mm Hub:11 ↔ ISO 7045 H M3 x 12 - 4.8 - H:27
- Mate:1011: 8mm Hub:12 ↔ AASG06
- Mate:1018: 8mm Hub:12 ↔ ISO 7045 H M3 x 12 - 4.8 - H:29
- Mate:1019: 8mm Hub:12 ↔ ISO 7045 H M3 x 12 - 4.8 - H:28
- Mate:1020: 8mm Hub:12 ↔ ISO 7045 H M3 x 12 - 4.8 - H:30
- Mate:1027: ISO 4035 M5:10 ↔ ISO 4018 M5 x 40:3
- Mate:1065: 4mm mounting hub:3 ↔ ISO 7045 H M3 x 8 - 4.8 - H:22
- Mate:1066: 4mm mounting hub:3 ↔ ISO 7045 H M3 x 8 - 4.8 - H:23
- Mate:1067: 6mm Mounting Hub:1 ↔ AASG06
- Mate:1069: 6mm Mounting Hub:1 ↔ AASG06
- Mate:1076: AA035c:1 ↔ Steel Rod 8mm x 140mm:1
- Mate:1077: AA035c:1 ↔ AASG02
- Mate:1083: AA001c:1 ↔ TSINY TS-42GZ495:1
- Mate:1084: AA001c:1 ↔ TSINY TS-42GZ495:1
- Mate:1085: AA001c:1 ↔ TSINY TS-42GZ495:1
- Mate:1086: AA001c:1 ↔ TSINY TS-42GZ495:1
- Mate:1087: TSINY TS-42GZ495:1 ↔ 8mm Hub:10
- Mate:1088: AA006b:1 ↔ EMS22XXX-D28-LSX:1
- Mate:1089: AA006b:1 ↔ EMS22XXX-D28-LSX:1
- Angle:17 (90 deg): AA006b:1 ↔ EMS22XXX-D28-LSX:1
- Mate:1090: 6mm Mounting Hub:2 ↔ EMS22XXX-D28-LSX:1
- Mate:1091: 6mm Mounting Hub:2 ↔ EMS22XXX-D28-LSX:1
- Mate:1093: AA001c:1 ↔ EMS22XXX-D28-LSX:2
- Angle:18 (180 deg): AA001c:1 ↔ EMS22XXX-D28-LSX:2
- Mate:1095: AA001c:1 ↔ EMS22XXX-D28-LSX:2
- Mate:1097: AA010b:1 ↔ TSINY TS-42GZ495:2
- Mate:1098: AA010b:1 ↔ TSINY TS-42GZ495:2
- Angle:21 (0 deg): AA010b:1 ↔ EMS22XXX-D28-LSX:3
- Mate:1100: AA010b:1 ↔ EMS22XXX-D28-LSX:3
- Mate:1101: AA010b:1 ↔ TSINY TS-42GZ495:2
- Mate:1102: AA010b:1 ↔ TSINY TS-42GZ495:2
- Mate:1104: AA008d2:1 ↔ TSINY TS-42GZ495:3
- Mate:1106: AA008d2:1 ↔ EMS22XXX-D28-LSX:4
- Mate:1107: AA008d2:1 ↔ EMS22XXX-D28-LSX:4
- Angle:22 (0 deg): AA008d2:1 ↔ EMS22XXX-D28-LSX:4
- Mate:1113: AA008c:1 ↔ AA008d2:1
- Mate:1114: AA008c:1 ↔ AA008d2:1
- Mate:1115: AA008c:1 ↔ AA008d2:1
- Mate:1117: TSINY TS-42GZ495:3 ↔ 6mm Mounting Hub:1
- Mate:1122: AA001c:1 ↔ Steel Rod 8mm x 140mm:1
- Mate:1124: AA008d2:1 ↔ AASG06
- Mate:1125: AA008c:1 ↔ AA008d2:1
- Mate:1126: AA010b:1 ↔ EMS22XXX-D28-LSX:3
- Mate:1128: TSINY TS-42GZ495:2 ↔ AASG03
- Mate:1129: TSINY TS-42GZ495:2 ↔ 8mm Hub:13
- Mate:1130: AA010b:1 ↔ 8mm Hub:13
- Mate:1131: 8mm Hub:13 ↔ AASG03
- Mate:1132: 8mm Hub:12 ↔ 6mm x 160mm D Shaft:1
- Mate:1133: 8mm Hub:12 ↔ AASG06
- Mate:1134: AASG06 ↔ 6mm x 160mm D Shaft:1
- Mate:1135: TSINY TS-42GZ495:3 ↔ 6mm x 160mm D Shaft:1
- Mate:1136: 6mm Mounting Hub:1 ↔ AASG06
- Mate:1137: 8mm Hub:12 ↔ AASG06
- Mate:1138: 6mm Mounting Hub:1 ↔ ISO 7045 H M3 x 12 - 4.8 - H:30
- Mate:1139: 6mm Mounting Hub:1 ↔ ISO 7045 H M3 x 12 - 4.8 - H:29
- Mate:1140: 6mm Mounting Hub:1 ↔ ISO 7045 H M3 x 12 - 4.8 - H:28
- Mate:1141: 8mm Hub:12 ↔ ISO 7045 H M3 x 12 - 4.8 - H:31
- Mate:1142: 8mm Hub:12 ↔ ISO 7045 H M3 x 12 - 4.8 - H:32
- Mate:1143: 8mm Hub:12 ↔ ISO 7045 H M3 x 12 - 4.8 - H:33
- Mate:1144: 8mm Hub:12 ↔ ISO 7045 H M3 x 12 - 4.8 - H:33
- Mate:1145: 8mm Hub:12 ↔ ISO 7045 H M3 x 12 - 4.8 - H:31
- Mate:1146: 8mm Hub:12 ↔ ISO 7045 H M3 x 12 - 4.8 - H:32
- Flush:29: 6mm Mounting Hub:1 ↔ 6mm x 160mm D Shaft:1
- Mate:1147: 6mm Mounting Hub:4 ↔ 6mm x 160mm D Shaft:1
- Mate:1148: 6mm Mounting Hub:4 ↔ ISO 7045 H M3 x 12 - 4.8 - H:18
- Mate:1150: 6mm Mounting Hub:4 ↔ ISO 7045 H M3 x 12 - 4.8 - H:20
- Mate:1152: AA010b:1 ↔ 6mm Mounting Hub:4
- Mate:1157: AA008d2:1 ↔ ISO 4018 M5 x 25:29
- Mate:1158: AA008d2:1 ↔ ISO 4018 M5 x 25:32
- Mate:1159: AA008d2:1 ↔ ISO 4018 M5 x 25:29
- Mate:1160: AA008d2:1 ↔ TSINY TS-42GZ495:3
- Mate:1161: AA008d2:1 ↔ TSINY TS-42GZ495:3
- Mate:1162: AA008d2:1 ↔ ISO 4018 M5 x 40:1
- Mate:1163: AA008d2:1 ↔ ISO 4018 M5 x 40:2
- Mate:1164: AA008d2:1 ↔ ISO 4018 M5 x 40:4
- Mate:1165: AA008d2:1 ↔ ISO 4018 M5 x 40:3
- Mate:1166: AA008d2:1 ↔ ISO 4018 M5 x 40:2
- Mate:1167: AA035c:1 ↔ ISO 4035 M5:1
- Mate:1168: AA035c:1 ↔ ISO 4035 M5:1
- Mate:1169: AA035c:1 ↔ ISO 4018 M5 x 40:1
- Mate:1170: AA008d2:1 ↔ AA035c:1
- Mate:1171: AA035c:1 ↔ ISO 4018 M5 x 40:4
- Mate:1172: AA035c:1 ↔ ISO 4018 M5 x 40:3
- Mate:1173: AA035c:1 ↔ ISO 4035 M5:10
- Mate:1174: ISO 4035 M5:9 ↔ ISO 4018 M5 x 40:4
- Mate:1175: AA035c:1 ↔ ISO 4035 M5:9
- Angle:24 (0 deg): AA035c:1 ↔ ISO 4035 M5:9
- Angle:25 (0 deg): AA035c:1 ↔ ISO 4035 M5:10
- Mate:1176: AA035c:1 ↔ ISO 4035 M5:2
- Flush:35: Steel Rod 8mm x 140mm:1 ↔ 8mm Hub:4
- Mate:1177: 6mm Mounting Hub:5 ↔ EMS22XXX-D28-LSX:2
- Mate:1178: 6mm Mounting Hub:5 ↔ AASG04
- Mate:1179: 6mm Mounting Hub:5 ↔ AASG04
- Mate:1180: EMS22XXX-D28-LSX:2 ↔ AASG04
- Mate:1181: 6mm Mounting Hub:6 ↔ EMS22XXX-D28-LSX:1
- Mate:1182: EMS22XXX-D28-LSX:1 ↔ AASG05
- Mate:1183: 6mm Mounting Hub:6 ↔ AASG05
- Mate:1184: 6mm Mounting Hub:6 ↔ AASG05
- Mate:1185: 6mm Mounting Hub:7 ↔ EMS22XXX-D28-LSX:3
- Mate:1186: 6mm Mounting Hub:7 ↔ AASG07
- Mate:1187: EMS22XXX-D28-LSX:3 ↔ AASG07
- Mate:1188: 6mm Mounting Hub:7 ↔ AASG07
- Mate:1189: 6mm Mounting Hub:8 ↔ EMS22XXX-D28-LSX:4
- Mate:1190: EMS22XXX-D28-LSX:4 ↔ AASG06
- Mate:1191: 6mm Mounting Hub:8 ↔ AASG06
- Mate:1192: AA008d2:1 ↔ ISO 4018 M5 x 25:30
- Mate:1193: AA008d2:1 ↔ ISO 4018 M5 x 25:30
- Mate:1194: AA008d2:1 ↔ ISO 4018 M5 x 25:31
- Mate:1195: AA008d2:1 ↔ ISO 4018 M5 x 25:31
- Mate:1196: AA051:1 ↔ Steel Rod 8mm x 110mm:1
- Mate:1197: AA036:1 ↔ AA051:1
- Mate:1198: AA036:1 ↔ 8mm Hub:14
- Mate:1199: AA036:1 ↔ 8mm Hub:14
- Mate:1200: AA036:1 ↔ 8mm Hub:14
- Mate:1201: AA052:1 ↔ Steel Rod 8mm x 140mm:1
- Mate:1202: AA035c:1 ↔ AA052:1
- Mate:1203: AA035c:1 ↔ 8mm Hub:6
- Mate:1204: AA010b:1 ↔ Steel Rod 8mm x 110mm:1
- Mate:1206: AA016b:1 ↔ EMS22XXX-D28-LSX:5
- Mate:1207: AA016b:1 ↔ EMS22XXX-D28-LSX:5
- Angle:26 (180 deg): AA016b:1 ↔ EMS22XXX-D28-LSX:5
- Mate:1208: 6mm Mounting Hub:9 ↔ EMS22XXX-D28-LSX:5
- Flush:36: 6mm Mounting Hub:9 ↔ 8mm Hub:7
- Mate:1209: 6mm Mounting Hub:9 ↔ AASG08
- Mate:1210: EMS22XXX-D28-LSX:5 ↔ AASG08
- Mate:1211: AA045b:1 ↔ EMS22XXX-D28-LSX:6
- Mate:1212: AA045b:1 ↔ EMS22XXX-D28-LSX:6
- Angle:27 (0 deg): AA045b:1 ↔ EMS22XXX-D28-LSX:6
- Mate:1213: AA034:1 ↔ AA045b:1
- Mate:1214: AA045b:1 ↔ ISO 4018 M5 x 25:41
- Mate:1215: AA045b:1 ↔ ISO 4018 M5 x 25:43
- Mate:1216: AA045b:1 ↔ Steel Rod 8mm x 80mm:1
- Mate:1217 (1 mm): AA045b:1 ↔ AA046:1
- Mate:1218: AA045b:1 ↔ AA049:1
- Mate:1219: AA045b:1 ↔ ISO 4018 M5 x 10:5
- Flush:37 (-2.5 mm): AA045b:1 ↔ Steel Rod 8mm x 80mm:1
- Mate:1220: 8mm Hub:8 ↔ AASG10
- Mate:1221: AA045b:1 ↔ AASG10
- Mate:1222: EMS22XXX-D28-LSX:6 ↔ AASG10
- Mate:1223: AA045b:1 ↔ AASG09
- Mate:1224: AA045b:1 ↔ 12V DC Motor 378-1:3
- Mate:1225: AA045b:1 ↔ 12V DC Motor 378-1:3
- Mate:1226: 4mm mounting hub:8 ↔ AASG09
- Mate:1227: AA045b:1 ↔ AASG09
- Mate:1228: EMS22XXX-D28-LSX:6 ↔ 6mm Mounting Hub:10
- Mate:1229: AASG10 ↔ 6mm Mounting Hub:10
- Mate:1230: QS12MM250:1 ↔ AASG05
- Mate:1232: EMS22XXX-D28-LSX:1 ↔ AASG05
- Mate:1233: AA006b:1 ↔ AASG05
- Mate:1234: Steel Rod 8mm x 80mm:1 ↔ 8mm Hub:8
- Mate:1235: AA045b:1 ↔ AASG10
- Mate:1236: 6mm Mounting Hub:4 ↔ ISO 7045 H M3 x 12 - 4.8 - H:19
- Mate:1237: AA010b:1 ↔ ISO 7045 H M3 x 12 - 4.8 - H:19
- Mate:1238: 6mm Mounting Hub:4 ↔ ISO 7045 H M3 x 12 - 4.8 - H:19
- Mate:1239: 6mm Mounting Hub:4 ↔ ISO 7045 H M3 x 12 - 4.8 - H:20
- Mate:1240: 6mm Mounting Hub:4 ↔ ISO 7045 H M3 x 12 - 4.8 - H:18
- Mate:1241: 6mm Mounting Hub:4 ↔ 6mm x 160mm D Shaft:1
- Mate:1242: 6mm Mounting Hub:4 ↔ 6mm x 160mm D Shaft:1
- Mate:1243: 6mm Mounting Hub:1 ↔ 6mm x 160mm D Shaft:1
- Mate:1244: 6mm Mounting Hub:1 ↔ 6mm x 160mm D Shaft:1
- Mate:1245: 8mm Hub:11 ↔ 6mm x 120mm D Shaft:1
- Mate:1247: 22x8x8mm Bearing:7 ↔ 6mm x 120mm D Shaft:1
- Mate:1248: 8mm Hub:7 ↔ 6mm x 120mm D Shaft:1
- Mate:1249: 8mm Hub:2 ↔ 6mm x 120mm D Shaft:1
- Mate:1250: AA041:1 ↔ 6mm x 120mm D Shaft:1
- Mate:1251: 4mm mounting hub:3 ↔ 6mm x 120mm D Shaft:1
- Mate:1252: 8mm Hub:11 ↔ 6mm x 120mm D Shaft:1
- Mate:1253: 8mm Hub:11 ↔ 6mm x 120mm D Shaft:1
- Mate:1254: 8mm Hub:2 ↔ 6mm x 120mm D Shaft:1
- Mate:1255: 8mm Hub:2 ↔ 6mm x 120mm D Shaft:1
- Mate:1256: AA034:1 ↔ ISO 7045 H M3 x 8 - 4.8 - H:30
- Mate:1257: AA034:1 ↔ 6mm x 120mm D Shaft:1
- Mate:1258: AA010b:1 ↔ AA053:1
- Mate:1259: AA010b:1 ↔ AA053:1
- Mate:1260 (0.5 mm): AA010b:1 ↔ AA053:1
- Mate:1261: AA001c:1 ↔ AA053:3
- Mate:1262: AA001c:1 ↔ AA053:3
- Mate:1263 (0.5 mm): AA001c:1 ↔ AA053:3
- Mate:1264: AA045b:1 ↔ 22x8x8mm Bearing:6
- Mate:1265: AA045b:1 ↔ 22x8x8mm Bearing:5
